# Autodesk Inventor assembly: Ensamble
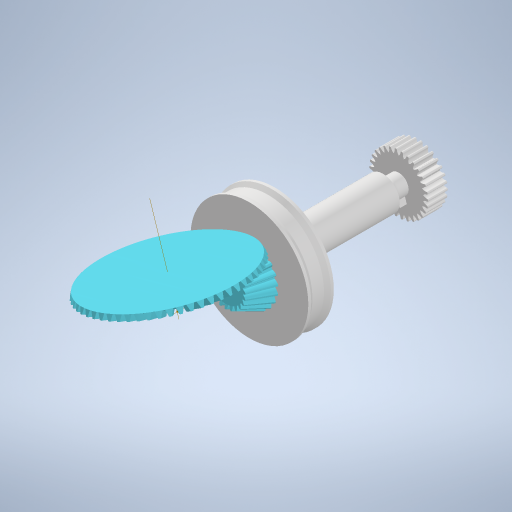
[picture p0: Inventor's stored thumbnail of the model, 512x512]
Saved by Autodesk Inventor 2024 (Build 280153000, 153)
## iProperties
Created: 2024-03-20
Part Number: Ensamble
Document SubType Name: Assembly
Designer: mater
Author: mater
## Documents named in this file (6)
- C:\Users\mater\OneDrive\Escritorio\U\5to ciclo\Dinamica Lab\Ensamble.iam
- C:\Users\mater\Downloads\EJE_CUÑEROS.ipt
- C:\Users\mater\Downloads\POLEA.ipt
- C:\Users\mater\Downloads\ENGRANE.ipt
- C:\Users\mater\Downloads\CUÑA.ipt
- C:\Users\mater\OneDrive\Escritorio\U\5to ciclo\Dinamica Lab\Ensamble\Design Accelerator\Bevel Gears1.iam
## Components (6 placed, 5 different names)
1. EJE_CUÑEROS:1 — Rigid:1, Flush:1, Rigid:2, Rigid:3, Rotational:1, Rigid:4
2. POLEA:1 — Rigid:1, Flush:1
3. CUÑA:1 — Rigid:2
4. ENGRANE:1 — Rigid:3
5. Bevel Gears:1 [sub-assembly] — Rotational:1
6. CUÑA:3 — Rigid:4
## Relationships (6: WeldJoint 4, Flush 1, RevoluteJoint 1)
- Rigid:1 [WeldJoint]: EJE_CUÑEROS:1 ↔ POLEA:1
- Flush:1: EJE_CUÑEROS:1 ↔ POLEA:1
- Rigid:2 [WeldJoint]: EJE_CUÑEROS:1 ↔ CUÑA:1
- Rigid:3 [WeldJoint]: EJE_CUÑEROS:1 ↔ ENGRANE:1
- Rotational:1 [RevoluteJoint]: EJE_CUÑEROS:1 ↔ Bevel Gears:1
- Rigid:4 [WeldJoint]: EJE_CUÑEROS:1 ↔ CUÑA:3
